# Autodesk Inventor assembly: Robotic Arm 3D Model
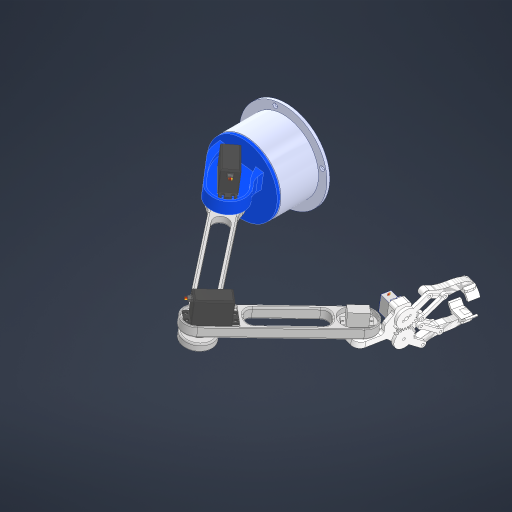
[picture p0: Inventor's stored thumbnail of the model, 512x512]
Saved by Autodesk Inventor 2024 (Build 280153000, 153)
## iProperties
Company: Unknown organisation
Created: 2023-03-04
Part Number: Robotic Arm 3D Model
Description: HOOPS Exchange Step
Document SubType Name: Assembly
Designer: hrush
Authority: Unknown authorisation
Sending System: HOOPS Exchange
Preprocessor: HOOPS Exchange 2022.1
Title: /tmp/filefZVxeh/Robotic Arm 3D Model.step
Author: root
## Documents named in this file (8)
- C:\CAD\Robotic Arm 3D Model step\Robotic Arm 3D Model.iam
- C:\CAD\Robotic Arm 3D Model step\Gripper Assembly.iam
- C:\CAD\Robotic Arm 3D Model step\Servo Motor Micro  9g.ipt
- C:\CAD\Robotic Arm 3D Model step\Servo Motor MG996R.ipt
- C:\CAD\Robotic Arm 3D Model step\Waist.ipt
- C:\CAD\Robotic Arm 3D Model step\Base.ipt
- C:\CAD\Robotic Arm 3D Model step\Arm 01-large.ipt
- C:\CAD\Robotic Arm 3D Model step\Arm 02-large.ipt
## Components (9 placed, 9 different names)
1. Gripper Assembly_1 [sub-assembly] — Rotational:3
2. Servo Motor MG996R_13 — Mate:10, Mate:11, Mate:12, Rotational:2
3. Waist_17 — Mate:4, Mate:5, Mate:7, Mate:8, Mate:9
4. Servo Motor Micro  9g_18 — Mate:13, Mate:14, Mate:15, Rotational:3
5. Base_19 — Mate:1, Mate:2, Mate:3
6. Servo Motor MG996R_20 — Mate:7, Mate:8, Mate:9, Rotational:1
7. Servo Motor MG996R_21 — Mate:1, Mate:2, Mate:3, Mate:4, Mate:5
8. Arm 01-large:1 — Rotational:1, Rotational:2
9. Arm 02-large:1 — Mate:10, Mate:11, Mate:12, Mate:13, Mate:14, Mate:15
## Relationships (17: Mate 14, RevoluteJoint 3)
- Mate:1: Base_19 ↔ Servo Motor MG996R_21
- Mate:2: Base_19 ↔ Servo Motor MG996R_21
- Mate:3: Base_19 ↔ Servo Motor MG996R_21
- Mate:4: Waist_17 ↔ Servo Motor MG996R_21
- Mate:5: Waist_17 ↔ Servo Motor MG996R_21
- Mate:7: Waist_17 ↔ Servo Motor MG996R_20
- Mate:8: Waist_17 ↔ Servo Motor MG996R_20
- Mate:9: Waist_17 ↔ Servo Motor MG996R_20
- Rotational:1 [RevoluteJoint]: Servo Motor MG996R_20 ↔ Arm 01-large:1
- Mate:10: Servo Motor MG996R_13 ↔ Arm 02-large:1
- Mate:11: Servo Motor MG996R_13 ↔ Arm 02-large:1
- Mate:12: Servo Motor MG996R_13 ↔ Arm 02-large:1
- Rotational:2 [RevoluteJoint]: Servo Motor MG996R_13 ↔ Arm 01-large:1
- Mate:13: Servo Motor Micro  9g_18 ↔ Arm 02-large:1
- Mate:14: Servo Motor Micro  9g_18 ↔ Arm 02-large:1
- Mate:15: Servo Motor Micro  9g_18 ↔ Arm 02-large:1
- Rotational:3 [RevoluteJoint]: Gripper Assembly_1 ↔ Servo Motor Micro  9g_18
